# Autodesk Inventor assembly: 3-finger_gripper_finger_B
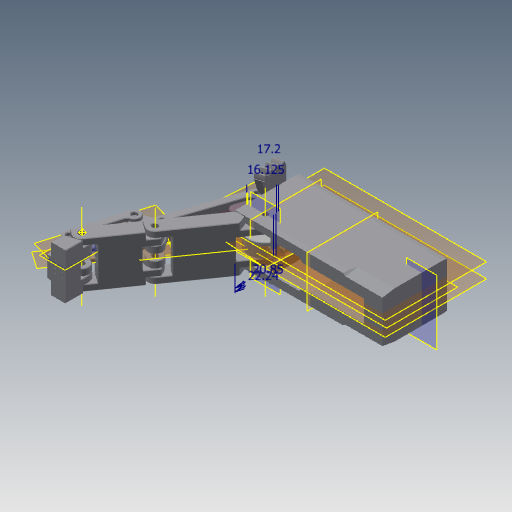
[picture p0: Inventor's stored thumbnail of the model, 512x512]
Saved by Autodesk Inventor 2018 (Build 220112000, 112)
## iProperties
Created: 2019-01-30
Part Number: 3-finger_gripper_finger_B
Document SubType Name: Assembly
Designer: Tsche
Author: Tsche
## Documents named in this file (17)
- C:\Users\Tsche\Documents\3d-printer\parts\grippers\Three_Finger_Gripper\BetaBots-Robot-Arm-Project-master\BetaBots-Robot-Arm-Project-master\ThreeFingerGripper\inventor\Gripper\3-finger_gripper_finger_B.iam
- C:\Users\Tsche\Documents\3d-printer\parts\grippers\Three_Finger_Gripper\BetaBots-Robot-Arm-Project-master\BetaBots-Robot-Arm-Project-master\ThreeFingerGripper\inventor\Gripper\finger_part_a.ipt
- C:\Users\Tsche\Documents\3d-printer\parts\grippers\Three_Finger_Gripper\BetaBots-Robot-Arm-Project-master\BetaBots-Robot-Arm-Project-master\ThreeFingerGripper\inventor\Gripper\finger_part_b.ipt
- C:\Users\Tsche\Documents\3d-printer\parts\grippers\Three_Finger_Gripper\BetaBots-Robot-Arm-Project-master\BetaBots-Robot-Arm-Project-master\ThreeFingerGripper\inventor\Gripper\finger_part_c.ipt
- C:\Users\Tsche\Documents\3d-printer\parts\grippers\Three_Finger_Gripper\BetaBots-Robot-Arm-Project-master\BetaBots-Robot-Arm-Project-master\ThreeFingerGripper\inventor\Gripper\bar_bc.ipt
- C:\Users\Tsche\Documents\3d-printer\parts\grippers\Three_Finger_Gripper\BetaBots-Robot-Arm-Project-master\BetaBots-Robot-Arm-Project-master\ThreeFingerGripper\inventor\Gripper\hinge_act_b.ipt
- C:\Users\Tsche\Documents\3d-printer\parts\grippers\Three_Finger_Gripper\BetaBots-Robot-Arm-Project-master\BetaBots-Robot-Arm-Project-master\ThreeFingerGripper\inventor\Gripper\bar_act_ab.ipt
- C:\Users\Tsche\Documents\3d-printer\parts\grippers\Three_Finger_Gripper\BetaBots-Robot-Arm-Project-master\BetaBots-Robot-Arm-Project-master\ThreeFingerGripper\inventor\Gripper\hinge_guid_b.ipt
- C:\Users\Tsche\Documents\3d-printer\parts\grippers\Three_Finger_Gripper\BetaBots-Robot-Arm-Project-master\BetaBots-Robot-Arm-Project-master\ThreeFingerGripper\inventor\Gripper\bar_guid_ab.ipt
- C:\Users\Tsche\Documents\3d-printer\parts\grippers\Three_Finger_Gripper\BetaBots-Robot-Arm-Project-master\BetaBots-Robot-Arm-Project-master\ThreeFingerGripper\inventor\Gripper\hinge_guid_a.ipt
- C:\Users\Tsche\Documents\3d-printer\parts\grippers\Three_Finger_Gripper\BetaBots-Robot-Arm-Project-master\BetaBots-Robot-Arm-Project-master\ThreeFingerGripper\inventor\Gripper\hinge_guid_c.ipt
- C:\Users\Tsche\Documents\3d-printer\parts\grippers\Three_Finger_Gripper\BetaBots-Robot-Arm-Project-master\BetaBots-Robot-Arm-Project-master\ThreeFingerGripper\inventor\Gripper\hinge_act_a2.ipt
- C:\Users\Tsche\Documents\3d-printer\parts\grippers\Three_Finger_Gripper\BetaBots-Robot-Arm-Project-master\BetaBots-Robot-Arm-Project-master\ThreeFingerGripper\inventor\Gripper\finger-main_base.ipt
- C:\Users\Tsche\Documents\3d-printer\parts\grippers\Three_Finger_Gripper\BetaBots-Robot-Arm-Project-master\BetaBots-Robot-Arm-Project-master\ThreeFingerGripper\inventor\Gripper\worm.ipt
- C:\Users\Tsche\Documents\3d-printer\parts\grippers\Three_Finger_Gripper\BetaBots-Robot-Arm-Project-master\BetaBots-Robot-Arm-Project-master\ThreeFingerGripper\inventor\Gripper\dc-motor_12V_60U-min.ipt
- C:\Users\Tsche\Documents\3d-printer\parts\grippers\Three_Finger_Gripper\BetaBots-Robot-Arm-Project-master\BetaBots-Robot-Arm-Project-master\ThreeFingerGripper\inventor\Gripper\tilt-gear_B.ipt
- C:\Users\Tsche\Documents\3d-printer\parts\grippers\Three_Finger_Gripper\BetaBots-Robot-Arm-Project-master\BetaBots-Robot-Arm-Project-master\ThreeFingerGripper\inventor\Gripper\Dimensions.xlsx
## Components (16 placed, 15 different names)
1. finger-main_base:1 — Cylindrical:20, Flush:12, Cylindrical:21, Mate:15, Angle:1, Mate:16, Mate:17, Flush:20
2. finger_part_a:1 — Cylindrical:1, Flush:1, Cylindrical:16, Cylindrical:19, Cylindrical:20, Flush:12, Mate:14
3. finger_part_b:1 — Cylindrical:1, Flush:1, Cylindrical:2, Mate:3, Cylindrical:4, Cylindrical:9
4. finger_part_c:1 — Cylindrical:2, Mate:3, Mate:4, Cylindrical:3, Cylindrical:14
5. bar_bc:1 — Mate:4, Cylindrical:3, Mate:5, Cylindrical:5, Mate:6, Flush:2
6. hinge_act_b:1 — Mate:5, Cylindrical:4, Cylindrical:5, Cylindrical:6
7. bar_act_ab:1 — Mate:6, Cylindrical:6, Mate:13, Cylindrical:18
8. bar_bc:2 — Flush:2, Mate:8, Cylindrical:10, Mate:11, Cylindrical:15
9. hinge_guid_b:1 — Mate:8, Cylindrical:9, Cylindrical:10, Mate:9, Cylindrical:11
10. bar_guid_ab:1 — Mate:9, Cylindrical:11, Flush:11, Cylindrical:17
11. hinge_guid_a:1 — Flush:11, Cylindrical:16, Cylindrical:17
12. hinge_guid_c:1 — Mate:11, Cylindrical:14, Cylindrical:15
13. Worm Gear:1 — Mate:13, Cylindrical:18, Cylindrical:19
14. Worm:2 — Cylindrical:21, Mate:14
15. dc-motor_12V_60U-min:1 — Mate:15, Angle:1, Mate:16
16. tilt-gear_B:1 — Mate:17, Mate:18, Flush:20, Mate:19
## Relationships (37: CylindricalJoint 17, Mate 14, Flush 5, Angle 1)
- Cylindrical:1: finger_part_a:1 ↔ finger_part_b:1
- Flush:1: finger_part_a:1 ↔ finger_part_b:1
- Cylindrical:2: finger_part_b:1 ↔ finger_part_c:1
- Mate:3: finger_part_b:1 ↔ finger_part_c:1
- Mate:4: finger_part_c:1 ↔ bar_bc:1
- Cylindrical:3: finger_part_c:1 ↔ bar_bc:1
- Mate:5: bar_bc:1 ↔ hinge_act_b:1
- Cylindrical:4: finger_part_b:1 ↔ hinge_act_b:1
- Cylindrical:5: bar_bc:1 ↔ hinge_act_b:1
- Mate:6: bar_bc:1 ↔ bar_act_ab:1
- Cylindrical:6: hinge_act_b:1 ↔ bar_act_ab:1
- Flush:2 (8 mm): bar_bc:1 ↔ bar_bc:2
- Mate:8: bar_bc:2 ↔ hinge_guid_b:1
- Cylindrical:9: finger_part_b:1 ↔ hinge_guid_b:1
- Cylindrical:10: bar_bc:2 ↔ hinge_guid_b:1
- Mate:9: hinge_guid_b:1 ↔ bar_guid_ab:1
- Cylindrical:11: hinge_guid_b:1 ↔ bar_guid_ab:1
- Flush:11: bar_guid_ab:1 ↔ hinge_guid_a:1
- Mate:11: bar_bc:2 ↔ hinge_guid_c:1
- Cylindrical:14: finger_part_c:1 ↔ hinge_guid_c:1
- Cylindrical:15: bar_bc:2 ↔ hinge_guid_c:1
- Cylindrical:16: finger_part_a:1 ↔ hinge_guid_a:1
- Cylindrical:17: bar_guid_ab:1 ↔ hinge_guid_a:1
- Mate:13: bar_act_ab:1 ↔ Worm Gear:1
- Cylindrical:18: bar_act_ab:1 ↔ Worm Gear:1
- Cylindrical:19: finger_part_a:1 ↔ Worm Gear:1
- Cylindrical:20: finger-main_base:1 ↔ finger_part_a:1
- Flush:12: finger-main_base:1 ↔ finger_part_a:1
- Cylindrical:21: finger-main_base:1 ↔ Worm:2
- Mate:14: finger_part_a:1 ↔ Worm:2
- Mate:15: finger-main_base:1 ↔ dc-motor_12V_60U-min:1
- Angle:1 (0 deg): finger-main_base:1 ↔ dc-motor_12V_60U-min:1
- Mate:16: finger-main_base:1 ↔ dc-motor_12V_60U-min:1
- Mate:17: finger-main_base:1 ↔ tilt-gear_B:1
- Mate:18: tilt-gear_B:1
- Flush:20 (-18.5 mm): finger-main_base:1 ↔ tilt-gear_B:1
- Mate:19: tilt-gear_B:1
## Named parameters: finger_width = 25 mm, finger_thickness = 8 mm, finger_part_A_length = 42.8625 mm, finger_part_B_length = 28.575 mm, finger_link_width = 3.5 mm, finger_link_clearence = 0.15 mm, tol = 0.075 mm, link_tol = 0.254 mm, bore_press = 3 mm, bore_clearance = 3.1 mm, bar_diameter = 6.5 mm, bar_thickness = 4 mm, bar_width = 7 mm, hinge_dist_sym_plane = 4 mm, hinge_thickness = 3 mm, hinge_act_length_c = 7.62 mm, hinge_act_length_bc = 16.66875 mm, hinge_act_length_ab = 11.049 mm, hinge_act_length_a = 21.43125 mm, hinge_guid_length_c = 9.525 mm, hinge_guid_length_bc = 9.525 mm, hinge_guid_length_ab = 17.145 mm, hinge_guid_length_a = 17.145 mm, bar_length_bc = 28.575 mm, bar_act_length_ab = 40.48125 mm, bar_guid_length_ab = 43.275 mm, champfer = 0.3 mm, fillet = 0.4 mm, gear_diameter = 14 mm, dist_finger_BC = 56.5 mm, dist_hinge_points = 56.5 mm, hinge_point = 16.5 mm
